# Autodesk Inventor assembly: MAINASSEMBLY
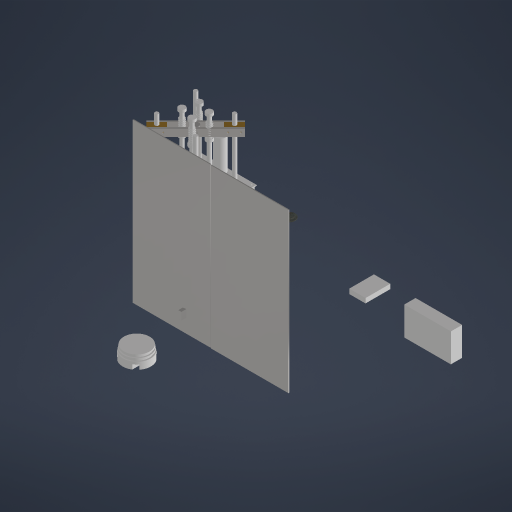
[picture p0: Inventor's stored thumbnail of the model, 512x512]
Saved by Autodesk Inventor 2024 (Build 280153000, 153)
## iProperties
Created: 2025-02-06
Part Number: MAINASSEMBLY
Document SubType Name: Assembly
Designer: Tommy Rohmann
Author: Tommy Rohmann
## Documents named in this file (16)
- C:\Users\Tommy Rohmann\OneDrive\Projects\Microgravity-Press-Washing-Machine\System Design and Documentation\Inventor Design Project\MAINASSEMBLY.iam
- C:\Users\Tommy Rohmann\OneDrive\Projects\Microgravity-Press-Washing-Machine\System Design and Documentation\Inventor Design Project\SUBWashChamber.iam
- C:\Users\Tommy Rohmann\OneDrive\Projects\Microgravity-Press-Washing-Machine\System Design and Documentation\Inventor Design Project\Actuated Ball Valves\SUBBallValve.iam
- C:\Users\Tommy Rohmann\OneDrive\Projects\Microgravity-Press-Washing-Machine\System Design and Documentation\Inventor Design Project\SUBReserviorPiston.iam
- C:\Users\Tommy Rohmann\OneDrive\Projects\Microgravity-Press-Washing-Machine\System Design and Documentation\Inventor Design Project\SUBConduitHatch.iam
- C:\Users\Tommy Rohmann\OneDrive\Projects\Microgravity-Press-Washing-Machine\System Design and Documentation\Inventor Design Project\.25inFittings\5779K109_Push-to-Connect Tube Fitting for Air .ipt
- C:\Users\Tommy Rohmann\OneDrive\Projects\Microgravity-Press-Washing-Machine\System Design and Documentation\Inventor Design Project\SUBFrameBottom.iam
- C:\Users\Tommy Rohmann\OneDrive\Projects\Microgravity-Press-Washing-Machine\System Design and Documentation\Inventor Design Project\SUBDriveShaftACME.iam
- C:\Users\Tommy Rohmann\OneDrive\Projects\Microgravity-Press-Washing-Machine\System Design and Documentation\Inventor Design Project\SUBWashPiston.iam
- C:\Users\Tommy Rohmann\OneDrive\Projects\Microgravity-Press-Washing-Machine\System Design and Documentation\Inventor Design Project\TensionerSprocket.ipt
- C:\Users\Tommy Rohmann\OneDrive\Projects\Microgravity-Press-Washing-Machine\System Design and Documentation\Inventor Design Project\SUBWashThrustArm.iam
- C:\Users\Tommy Rohmann\OneDrive\Projects\Microgravity-Press-Washing-Machine\System Design and Documentation\Inventor Design Project\LCDScreen.ipt
- C:\Users\Tommy Rohmann\OneDrive\Projects\Microgravity-Press-Washing-Machine\System Design and Documentation\Inventor Design Project\PowerSupply.ipt
- C:\Users\Tommy Rohmann\OneDrive\Projects\Microgravity-Press-Washing-Machine\System Design and Documentation\Inventor Design Project\RaspberryPi.ipt
- C:\Users\Tommy Rohmann\OneDrive\Projects\Microgravity-Press-Washing-Machine\System Design and Documentation\Inventor Design Project\SUBSuperStructure.iam
- C:\Users\Tommy Rohmann\OneDrive\Projects\Microgravity-Press-Washing-Machine\System Design and Documentation\Inventor Design Project\DriveTrainBase.iam
## Components (20 placed, 15 different names)
1. SUBWashChamber:1 [sub-assembly] — Mate:1, Tangent:1, Mate:4, Mate:5, Mate:9, Mate:10, Mate:11, Mate:12, Mate:14, Mate:27
2. SUBBallValve:1 [sub-assembly] — Mate:26, Flush:3
3. SUBReserviorPiston:1 [sub-assembly] — Mate:4
4. SUBConduitHatch:1 [sub-assembly]
5. 5779K109_Push-to-Connect Tube Fitting for Air :1 — Mate:1, Tangent:1
6. SUBFrameBottom:1 [sub-assembly] — Mate:9, Mate:12
7. SUBWashPiston:1 [sub-assembly] — Mate:5, Mate:6, Flush:1, Tangent:2
8. TensionerSprocket:1
9. SUBWashThrustArm:1 [sub-assembly] — Mate:6, Flush:1, Tangent:2, Mate:21
10. LCDScreen:1
11. PowerSupply:1
12. RaspberryPi:1
13. SUBFrameBottom:2 [sub-assembly] — Mate:10, Mate:11, Mate:25, Mate:26, Flush:3
14. SUBSuperStructure:1 [sub-assembly] — Mate:24, Mate:25, Flush:2
15. SUBSuperStructure:2 [sub-assembly]
16. DriveTrainBase:1 [sub-assembly] — Mate:14, Mate:15, Mate:16, Mate:17, Mate:18, Mate:19, Mate:20, Mate:22, Mate:23, Mate:24, Flush:2, Mate:27
17. SUBDriveShaftACME:1 [sub-assembly] — Mate:22, Mate:23
18. SUBDriveShaftACME:2 [sub-assembly] — Mate:17, Mate:18
19. SUBDriveShaftACME:3 [sub-assembly] — Mate:16, Mate:20
20. SUBDriveShaftACME:4 [sub-assembly] — Mate:15, Mate:19, Mate:21
## Relationships (27: Mate 22, Flush 3, Tangent 2)
- Mate:1: SUBWashChamber:1 ↔ 5779K109_Push-to-Connect Tube Fitting for Air :1
- Tangent:1 (10.16 mm): SUBWashChamber:1 ↔ 5779K109_Push-to-Connect Tube Fitting for Air :1
- Mate:4: SUBWashChamber:1 ↔ SUBReserviorPiston:1
- Mate:5: SUBWashChamber:1 ↔ SUBWashPiston:1
- Mate:6: SUBWashPiston:1 ↔ SUBWashThrustArm:1
- Flush:1: SUBWashPiston:1 ↔ SUBWashThrustArm:1
- Tangent:2: SUBWashPiston:1 ↔ SUBWashThrustArm:1
- Mate:9: SUBWashChamber:1 ↔ SUBFrameBottom:1
- Mate:10: SUBWashChamber:1 ↔ SUBFrameBottom:2
- Mate:11: SUBWashChamber:1 ↔ SUBFrameBottom:2
- Mate:12: SUBWashChamber:1 ↔ SUBFrameBottom:1
- Mate:14: SUBWashChamber:1 ↔ DriveTrainBase:1
- Mate:15: DriveTrainBase:1 ↔ SUBDriveShaftACME:4
- Mate:16: DriveTrainBase:1 ↔ SUBDriveShaftACME:3
- Mate:17: DriveTrainBase:1 ↔ SUBDriveShaftACME:2
- Mate:18: DriveTrainBase:1 ↔ SUBDriveShaftACME:2
- Mate:19: DriveTrainBase:1 ↔ SUBDriveShaftACME:4
- Mate:20: DriveTrainBase:1 ↔ SUBDriveShaftACME:3
- Mate:21: SUBWashThrustArm:1 ↔ SUBDriveShaftACME:4
- Mate:22: DriveTrainBase:1 ↔ SUBDriveShaftACME:1
- Mate:23: DriveTrainBase:1 ↔ SUBDriveShaftACME:1
- Mate:24: SUBSuperStructure:1 ↔ DriveTrainBase:1
- Mate:25: SUBFrameBottom:2 ↔ SUBSuperStructure:1
- Flush:2 (-3.175 mm): SUBSuperStructure:1 ↔ DriveTrainBase:1
- Mate:26: SUBBallValve:1 ↔ SUBFrameBottom:2
- Flush:3: SUBBallValve:1 ↔ SUBFrameBottom:2
- Mate:27: SUBWashChamber:1 ↔ DriveTrainBase:1
